# Autodesk Inventor assembly: iPadHolderAssembly
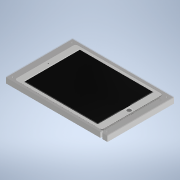
[picture p0: Inventor's stored thumbnail of the model, 180x180]
Saved by Autodesk Inventor 2021.1 (Build 251245010, 245A)
## iProperties
Created: 2020-11-06
Part Number: iPadHolderAssembly
Document SubType Name: Assembly
Designer: gisen
Author: gisen
## Documents named in this file (4)
- C:\Users\gisen\GitProjects\CAD-Data\CuboidAccessories\SecurityBox\Assemblies\iPadHolderAssembly.iam
- C:\Users\gisen\GitProjects\CAD-Data\CuboidAccessories\SecurityBox\3DPrintedParts\iPadHolder.ipt
- C:\Users\gisen\GitProjects\CAD-Data\Devices\iPad\iPadModelA2197.ipt
- C:\Users\gisen\GitProjects\CAD-Data\CuboidAccessories\SecurityBox\Plates\iPadCoverPlate.ipt
## Components (3 placed, 3 different names)
1. iPadHolder:1 — メイト:1, メイト:2, メイト:3, メイト:4, フラッシュ:1, フラッシュ:2
2. iPadModelA2197:1 — メイト:1, メイト:2, メイト:3
3. iPadCoverPlate:1 — メイト:4, フラッシュ:1, フラッシュ:2
## Relationships (6: Mate 4, Flush 2)
- メイト:1 [Mate]: iPadHolder:1 ↔ iPadModelA2197:1
- メイト:2 [Mate]: iPadHolder:1 ↔ iPadModelA2197:1
- メイト:3 [Mate]: iPadHolder:1 ↔ iPadModelA2197:1
- メイト:4 [Mate]: iPadHolder:1 ↔ iPadCoverPlate:1
- フラッシュ:1 [Flush]: iPadHolder:1 ↔ iPadCoverPlate:1
- フラッシュ:2 [Flush]: iPadHolder:1 ↔ iPadCoverPlate:1
